# Autodesk Inventor assembly: ASY GBK 3310 central wall shield 7
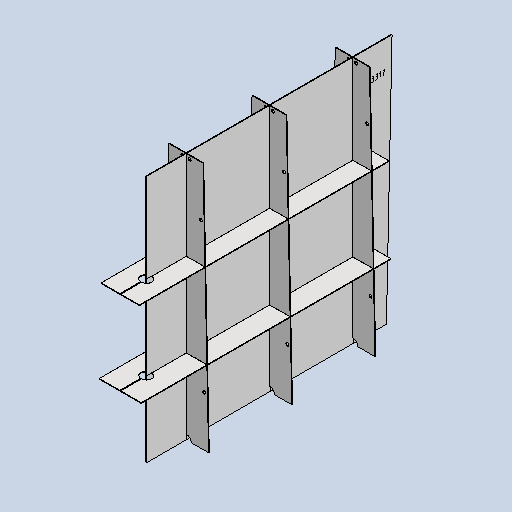
[picture p0: Inventor's stored thumbnail of the model, 512x512]
Saved by Autodesk Inventor 2026.2 (Build 302298010, 298A)
## iProperties
Created: 2026-05-19
Part Number: ASY GBK 3310 central wall shield 7
Document SubType Name: Assembly
Designer: pokla
Mass: 123029 g
Surface Area: 79995.2 cm^2
Volume: 15672.5 cm^3
Author: admin
## Documents named in this file (6)
- C:\Users\admin\Documents\Inventor\GBK-Gubkinskiy\ASY GBK 3310 central wall shield 7.iam
- C:\Users\admin\Documents\Inventor\GBK-Gubkinskiy\GBK 3312 stringer 7.ipt
- C:\Users\admin\Documents\Inventor\GBK-Gubkinskiy\GBK 3317 shield 7.ipt
- C:\Users\admin\Documents\Inventor\GBK-Gubkinskiy\GBK 3313 stringer 8.ipt
- C:\Users\admin\Documents\Inventor\GBK-Gubkinskiy\GBK 3311 central third rib.ipt
- C:\Users\admin\Documents\Inventor\GBK-Gubkinskiy\GBK 0101 main rib.ipt
## Components (11 placed, 5 different names)
1. GBK 3312 stringer 7.ipt:1 — Rigid:1
2. GBK 3317 shield 7.ipt:1 — Flush:7, Mate:5, Mate:2, Flush:1, Mate:1, Flush:6, Mate:4, Flush:6
3. GBK 3313 stringer 8.ipt:1 — Rigid:2, Rigid:7, Rigid:8
4. GBK 3312 stringer 7.ipt:2 — Rigid:4
5. GBK 3313 stringer 8.ipt:2 — Rigid:3, Rigid:5, Rigid:6, Flush:6
6. GBK 3311 central third rib.ipt:2 — Flush:7, Mate:5, Flush:4, Rigid:1, Rigid:2
7. GBK 3311 central third rib.ipt:1 — Flush:6, Flush:4, Mate:4, Rigid:4, Rigid:3
8. GBK 3311 central third rib:3 — Rigid:6
9. GBK 3311 central third rib:4 — Rigid:5
10. GBK 3311 central third rib:5 — Rigid:7
11. GBK 3311 central third rib:6 — Rigid:8
## Relationships (17: WeldJoint 8, Flush 5, Mate 4)
- Flush:7: GBK 3317 shield 7.ipt:1 ↔ GBK 3311 central third rib.ipt:2
- Mate:5: GBK 3317 shield 7.ipt:1 ↔ GBK 3311 central third rib.ipt:2
- Mate:2: GBK 3317 shield 7.ipt:1
- Flush:1: GBK 3317 shield 7.ipt:1
- Mate:1: GBK 3317 shield 7.ipt:1
- Flush:6: GBK 3317 shield 7.ipt:1 ↔ GBK 3311 central third rib.ipt:1
- Flush:4: GBK 3311 central third rib.ipt:2 ↔ GBK 3311 central third rib.ipt:1
- Mate:4: GBK 3317 shield 7.ipt:1 ↔ GBK 3311 central third rib.ipt:1
- Rigid:1 [WeldJoint] (4 mm): GBK 3312 stringer 7.ipt:1 ↔ GBK 3311 central third rib.ipt:2
- Rigid:2 [WeldJoint] (4 mm): GBK 3313 stringer 8.ipt:1 ↔ GBK 3311 central third rib.ipt:2
- Rigid:4 [WeldJoint] (4 mm): GBK 3312 stringer 7.ipt:2 ↔ GBK 3311 central third rib.ipt:1
- Rigid:3 [WeldJoint] (4 mm): GBK 3313 stringer 8.ipt:2 ↔ GBK 3311 central third rib.ipt:1
- Rigid:5 [WeldJoint] (4 mm): GBK 3313 stringer 8.ipt:2 ↔ GBK 3311 central third rib:4
- Rigid:6 [WeldJoint] (4 mm): GBK 3313 stringer 8.ipt:2 ↔ GBK 3311 central third rib:3
- Rigid:7 [WeldJoint] (4 mm): GBK 3313 stringer 8.ipt:1 ↔ GBK 3311 central third rib:5
- Rigid:8 [WeldJoint] (4 mm): GBK 3313 stringer 8.ipt:1 ↔ GBK 3311 central third rib:6
- Flush:6 (155 mm): GBK 3317 shield 7.ipt:1 ↔ GBK 3313 stringer 8.ipt:2
## Named parameters: Шаг_шпангоутов = 496.66667 mm
